# Autodesk Inventor assembly: modularRICH
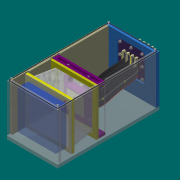
[picture p0: Inventor's stored thumbnail of the model, 180x180]
Saved by Autodesk Inventor 2016 SP1 (Build 200210100, 210)
## iProperties
Created: 2015-10-13
Part Number: modularRICH
Document SubType Name: Assembly
Designer: Sawaiz
Author: Sawaiz
## Documents named in this file (8)
- C:\Users\Sawaiz\OneDrive\projects\modularRICH\modularRICH.iam
- C:\Users\Sawaiz\OneDrive\projects\modularRICH\frame\frame.iam
- C:\Users\Sawaiz\OneDrive\projects\modularRICH\fresnelLens.ipt
- C:\Users\Sawaiz\OneDrive\projects\modularRICH\H12700A\H12700ASuppourt.iam
- C:\Users\Sawaiz\OneDrive\projects\modularRICH\aerogel\aerogelInHolder.iam
- C:\Users\Sawaiz\OneDrive\projects\modularRICH\mirror\mirrorHolder.iam
- C:\Users\Sawaiz\OneDrive\projects\modularRICH\modularRICH\AIP\Cable and Harness\modularRICH.Harness1.iam
- C:\Users\Sawaiz\OneDrive\projects\modularRICH\modularRICH.xlsx
## Components (6 placed, 6 different names)
1. frame:1 [sub-assembly] — Mate:20, Mate:21, Mate:26, Mate:28
2. H12700ASuppourt:1 [sub-assembly] — Mate:27, Mate:28, Flush:17
3. aerogelInHolder:1 [sub-assembly] — Flush:11, Flush:12, Mate:20, Mate:21, Mate:23, Flush:15, Flush:16, Mate:26
4. mirrorHolder:1 [sub-assembly] — Flush:11, Flush:12, Mate:24, Mate:27, Flush:17
5. fresnelLens:1 — Mate:23, Flush:15, Flush:16, Mate:24
6. Harness1 [sub-assembly]
## Relationships (12: Mate 7, Flush 5)
- Flush:11: aerogelInHolder:1 ↔ mirrorHolder:1
- Flush:12: aerogelInHolder:1 ↔ mirrorHolder:1
- Mate:20: frame:1 ↔ aerogelInHolder:1
- Mate:21: frame:1 ↔ aerogelInHolder:1
- Mate:23: aerogelInHolder:1 ↔ fresnelLens:1
- Flush:15: aerogelInHolder:1 ↔ fresnelLens:1
- Flush:16: aerogelInHolder:1 ↔ fresnelLens:1
- Mate:24: mirrorHolder:1 ↔ fresnelLens:1
- Mate:26: frame:1 ↔ aerogelInHolder:1
- Mate:27: H12700ASuppourt:1 ↔ mirrorHolder:1
- Mate:28: frame:1 ↔ H12700ASuppourt:1
- Flush:17: H12700ASuppourt:1 ↔ mirrorHolder:1
## Named parameters: acrylicThickness = 6.35 mm, aerogelThickness = 30 mm, height = 127 mm, width = 127 mm, depth = 273.05 mm, mirrorAngle = 5 deg, detectorWidth = 52 mm, detectorHeight = 52 mm, mirrorThickness = 3.175 mm, fresnelThickness = 0.1 mm, grooveDensity = 100, focalLength = 76.2 mm, ior = 1.49, centerThickness = 1.524 mm, fresnelAngle = 90 deg, fresnelEffectiveDiameter = 152.4 mm, mirrorSuppourtWidth = 38.1 mm, backGrooveBit = 4.8006 mm, sensorHolderWidth = 88.9 mm, sensorHolderSesnorHeight = 53.975 mm, sensorHolderSensorWidth = 53.975 mm, sensorHolderHeight = 88.9 mm, sensorHolderSensorHeight = 53.975 mm, sensorHolderORingGroove = 3.175 mm, sensorHolderORing = 3.175 mm, sensorHolderFlushORingID = 304.8 mm, sensorHolderFlushORing = 3.175 mm, oRingWidth = 1.5875 mm, sensorHolderORingID = 203.2 mm, frontBackORingID = 419.1 mm, topBottomHorizontalMirrorGroove = 12.7 mm, backMirrorGroove = 6.35 mm, mirrorGroove = 19.05 mm, compressionPercent = 40, fresnelChamfer = 6.35 mm, mirrorGrooveFillet = 6.35 mm, mirrorGrooveDrill = 6.35 mm, mirrorGrooveMill = 3.175 mm, fresnelMirrorChamfer = 6.35 mm, detectorOpeningHeight = 76.2 mm, detectorOpeningWidth = 76.2 mm, sensorHolderDepth = 19.05 mm, aerogelHeight = 110 mm, aerogelWidth = 110 mm, frameAcrylicThickness = 9.525 mm, internalAcrylicThicnkess = 6.35 mm, internalAcrylicThickness = 6.35 mm, aerogelClearence = 3.175 mm, backplanePCBWidth = 76.2 mm, backplanePCBHeight = 76.2 mm, backplaneHoleOffsett = 6.35 mm, backplanePostionOffsett = 12.7 mm, moduleSlotClearence = 0.79375 mm, testMountWidth = 300 mm, testMountHeight = 300 mm, testMountLength = 500 mm
